# Autodesk Inventor assembly: 15mm-QS15-galvo-assembly
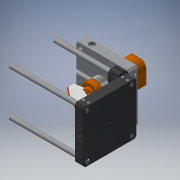
[picture p0: Inventor's stored thumbnail of the model, 180x180]
Saved by Autodesk Inventor 2017 (Build 210142000, 142)
## iProperties
Created: 2022-06-02
Part Number: 15mm-QS15-galvo-assembly
Document SubType Name: Assembly
Designer: Nikita
Author: Nikita
## Documents named in this file (7)
- C:\Users\Nikita\Documents\GitHub\mesoSPIM-bt-hardware\Benchtop\custom-parts\galvo-assembly\15mm-galvo(Thorlabs-QS15)-mount\15mm-QS15-galvo-assembly.iam
- C:\Users\Nikita\Documents\GitHub\mesoSPIM-bt-hardware\Benchtop\custom-parts\galvo-assembly\15mm-galvo(Thorlabs-QS15)-mount\QS15-mount-modified-Thorlabs-CagePlate-LCP03.ipt
- C:\Users\Nikita\Documents\GitHub\mesoSPIM-bt-hardware\Benchtop\custom-parts\CAD-library\Thorlabs\Galvos\Galvo-QS15X.ipt
- C:\Users\Nikita\Documents\GitHub\mesoSPIM-bt-hardware\Benchtop\custom-parts\CAD-library\Thorlabs\60mm_cage_system\LCP01B.ipt
- C:\Users\Nikita\Documents\GitHub\mesoSPIM-bt-hardware\Benchtop\custom-parts\CAD-library\Thorlabs\cage_rods\ER4_CageRod.ipt
- C:\Users\Nikita\Documents\GitHub\mesoSPIM-bt-hardware\Benchtop\custom-parts\CAD-library\Thorlabs\cage_rods\ER_CageRod.ipt
- C:\Users\Nikita\Documents\GitHub\mesoSPIM-bt-hardware\Benchtop\custom-parts\CAD-library\Thorlabs\60mm_cage_system\CagePlate-LCP03_M.ipt
## Components (8 placed, 5 different names)
1. QS15-mount-modified-Thorlabs-CagePlate-LCP03:1 — Insert:1, Angle:1, Angle:2
2. Galvo-QS15X:1
3. LCP01B:1 — Insert:1, Angle:1, Insert:2, Insert:3
4. ER4_CageRod:1 — Insert:2, Insert:4
5. ER4_CageRod:2 — Insert:3
6. ER4_CageRod:3 — Insert:5
7. ER4_CageRod:4 — Insert:6
8. CagePlate-LCP03_M:1 — Insert:4, Angle:2, Insert:5, Insert:6
## Relationships (8: Insert 6, Angle 2)
- Insert:1: QS15-mount-modified-Thorlabs-CagePlate-LCP03:1 ↔ LCP01B:1
- Angle:1 (0 deg): QS15-mount-modified-Thorlabs-CagePlate-LCP03:1 ↔ LCP01B:1
- Insert:2 (-10 mm): LCP01B:1 ↔ ER4_CageRod:1
- Insert:3 (-10 mm): LCP01B:1 ↔ ER4_CageRod:2
- Insert:4 (-10 mm): ER4_CageRod:1 ↔ CagePlate-LCP03_M:1
- Angle:2 (0 deg): QS15-mount-modified-Thorlabs-CagePlate-LCP03:1 ↔ CagePlate-LCP03_M:1
- Insert:5 (-10 mm): ER4_CageRod:3 ↔ CagePlate-LCP03_M:1
- Insert:6 (-10 mm): ER4_CageRod:4 ↔ CagePlate-LCP03_M:1
